# Autodesk Inventor assembly: TB_Fullassemb
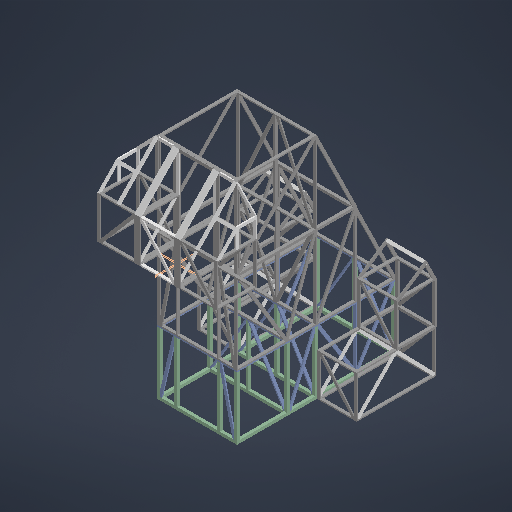
[picture p0: Inventor's stored thumbnail of the model, 512x512]
Saved by Autodesk Inventor 2026 (Build 300175000, 175)
## iProperties
Created: 2025-08-28
Part Number: TB_Fullassemb
Document SubType Name: Assembly
Designer: trott
Author: trott
## Documents named in this file (8)
- C:\Users\trott\Documents\UofSC-ASME-Tiger-Burn-Design-2025\CAD\Assembly\TB_Fullassemb.iam
- C:\Users\trott\Documents\UofSC-ASME-Tiger-Burn-Design-2025\CAD\Body\Base 01\Base 01.iam
- C:\Users\trott\Documents\UofSC-ASME-Tiger-Burn-Design-2025\CAD\Body\Base 02\Base 02.iam
- C:\Users\trott\Documents\UofSC-ASME-Tiger-Burn-Design-2025\CAD\Body\Base 03\Base 03.iam
- C:\Users\trott\Documents\UofSC-ASME-Tiger-Burn-Design-2025\CAD\Legs\Shoulder\Shoulder.iam
- C:\Users\trott\Documents\UofSC-ASME-Tiger-Burn-Design-2025\CAD\Legs\Shoulder\Shoulder_MIR.iam
- C:\Users\trott\Documents\UofSC-ASME-Tiger-Burn-Design-2025\CAD\Legs\Back Foot\B_Foot.iam
- C:\Users\trott\Documents\UofSC-ASME-Tiger-Burn-Design-2025\CAD\Legs\Back Leg\B_Legs0.iam
## Components (9 placed, 7 different names)
1. Base 01:1 [sub-assembly] — Mate:1, Flush:1, Flush:2, Flush:8, Mate:5, Flush:9, Mate:6, Flush:10, Flush:11, Flush:12, Mate:8, Flush:13
2. Base 02:1 [sub-assembly] — Mate:1, Flush:1, Flush:2, Mate:2, Flush:3, Flush:4
3. Base 03:1 [sub-assembly] — Mate:2, Flush:3, Flush:4, Flush:5, Flush:6, Mate:3, Mate:4, Flush:7
4. Shoulder:1 [sub-assembly] — Flush:5, Flush:6, Mate:3
5. Shoulder_MIR:1 [sub-assembly] — Mate:4, Flush:7
6. B_Foot:1 [sub-assembly] — Flush:8, Mate:5, Flush:9, Mate:7
7. B_Foot:2 [sub-assembly] — Mate:6, Flush:10, Flush:11, Mate:9
8. B_Legs0:1 [sub-assembly] — Mate:7, Flush:12, Mate:8
9. B_Legs0:2 [sub-assembly] — Mate:9, Flush:13
## Relationships (22: Flush 13, Mate 9)
- Mate:1: Base 01:1 ↔ Base 02:1
- Flush:1: Base 01:1 ↔ Base 02:1
- Flush:2: Base 01:1 ↔ Base 02:1
- Mate:2: Base 02:1 ↔ Base 03:1
- Flush:3: Base 02:1 ↔ Base 03:1
- Flush:4: Base 02:1 ↔ Base 03:1
- Flush:5: Base 03:1 ↔ Shoulder:1
- Flush:6: Base 03:1 ↔ Shoulder:1
- Mate:3: Base 03:1 ↔ Shoulder:1
- Mate:4: Base 03:1 ↔ Shoulder_MIR:1
- Flush:7: Base 03:1 ↔ Shoulder_MIR:1
- Flush:8: Base 01:1 ↔ B_Foot:1
- Mate:5: Base 01:1 ↔ B_Foot:1
- Flush:9: Base 01:1 ↔ B_Foot:1
- Mate:6: Base 01:1 ↔ B_Foot:2
- Flush:10: Base 01:1 ↔ B_Foot:2
- Flush:11: Base 01:1 ↔ B_Foot:2
- Mate:7: B_Foot:1 ↔ B_Legs0:1
- Flush:12: Base 01:1 ↔ B_Legs0:1
- Mate:8: Base 01:1 ↔ B_Legs0:1
- Mate:9: B_Foot:2 ↔ B_Legs0:2
- Flush:13: Base 01:1 ↔ B_Legs0:2
